# Autodesk Inventor assembly: HalfChassisAssem
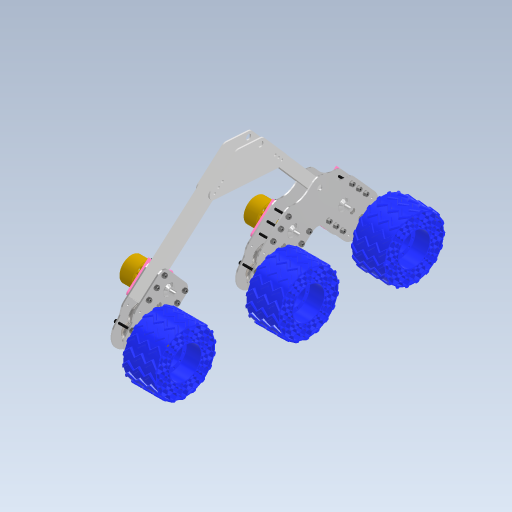
[picture p0: Inventor's stored thumbnail of the model, 512x512]
Saved by Autodesk Inventor 2023 (Build 270158000, 158)
## iProperties
Created: 2023-04-06
Part Number: HalfChassisAssem
Document SubType Name: Assembly
Designer: Dave
Author: Dave
## Documents named in this file (7)
- C:\Users\Dave\Documents\GitHub\BehrendURCMechanical\CAD\Chassis V3\HalfChassisAssem.iam
- C:\Users\Dave\Documents\GitHub\BehrendURCMechanical\CAD\Chassis V3\L3 Gearbox Assembly.iam
- C:\Users\Dave\Documents\GitHub\BehrendURCMechanical\CAD\Chassis V3\L1 Gearbox Assembly.iam
- C:\Users\Dave\Documents\GitHub\BehrendURCMechanical\CAD\Chassis V3\HipPivotPlate.ipt
- C:\Users\Dave\Documents\GitHub\BehrendURCMechanical\CAD\Chassis V3\aluminumextrusiontool.ipt
- C:\Users\Dave\Documents\GitHub\BehrendURCMechanical\CAD\Chassis V3\aluminumextrusiontool\aluminumextrusiontool-17-10.6in.ipt
- C:\Users\Dave\Documents\GitHub\BehrendURCMechanical\CAD\Chassis V3\aluminumextrusiontool\Part1-03.ipt
## Components (6 placed, 5 different names)
1. L3 Gearbox Assembly:1 [sub-assembly] — Flush:1, Mate:4, Tangent:2
2. L1 Gearbox Assembly:1 [sub-assembly] — Flush:1, Flush:2, Flush:3, Mate:1, Flush:6, Mate:2, Flush:7, Mate:3
3. HipPivotPlate:1 — Flush:3, Flush:4, Flush:5, Mate:5
4. HipPivotPlate:2 — Flush:2, Flush:4, Flush:5, Mate:1, Flush:6, Mate:4, Flush:8, Tangent:1, Mate:6, Flush:9
5. aluminumextrusiontool-17-10.6in:1 — Mate:2, Flush:7, Mate:3
6. Part1-03:2 — Mate:5, Flush:8, Tangent:1, Tangent:2
## Relationships (17: Flush 9, Mate 6, Tangent 2)
- Flush:1: L3 Gearbox Assembly:1 ↔ L1 Gearbox Assembly:1
- Flush:2: L1 Gearbox Assembly:1 ↔ HipPivotPlate:2
- Flush:3: L1 Gearbox Assembly:1 ↔ HipPivotPlate:1
- Flush:4: HipPivotPlate:1 ↔ HipPivotPlate:2
- Flush:5: HipPivotPlate:1 ↔ HipPivotPlate:2
- Mate:1 (396 mm): L1 Gearbox Assembly:1 ↔ HipPivotPlate:2
- Flush:6: L1 Gearbox Assembly:1 ↔ HipPivotPlate:2
- Mate:2: L1 Gearbox Assembly:1 ↔ aluminumextrusiontool-17-10.6in:1
- Flush:7: L1 Gearbox Assembly:1 ↔ aluminumextrusiontool-17-10.6in:1
- Mate:3 (-76.2 mm): L1 Gearbox Assembly:1 ↔ aluminumextrusiontool-17-10.6in:1
- Mate:4 (216 mm): L3 Gearbox Assembly:1 ↔ HipPivotPlate:2
- Mate:5: HipPivotPlate:1 ↔ Part1-03:2
- Flush:8: HipPivotPlate:2 ↔ Part1-03:2
- Tangent:1 (12.7 mm): HipPivotPlate:2 ↔ Part1-03:2
- Tangent:2 (6.35 mm): L3 Gearbox Assembly:1 ↔ Part1-03:2
- Mate:6: HipPivotPlate:2
- Flush:9: HipPivotPlate:2
